# Autodesk Inventor assembly: Assembly2
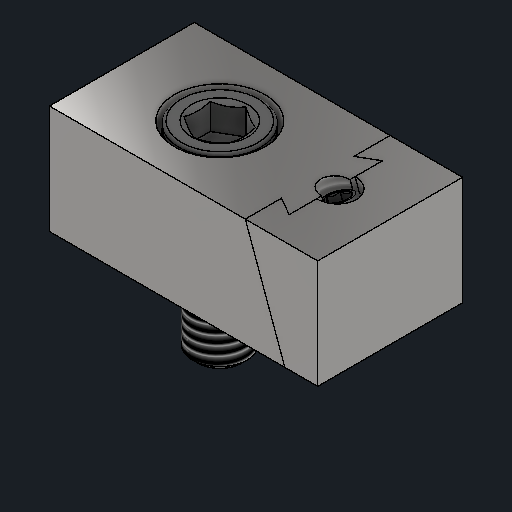
[picture p0: Inventor's stored thumbnail of the model, 512x512]
Saved by Autodesk Inventor 2026.2 (Build 302298000, 298)
## iProperties
Created: 2026-09-23
Part Number: Assembly2
Document SubType Name: Assembly
Designer: JoshuaEah
Author: JoshuaEah
## Documents named in this file (5)
- C:\Users\JoshuaEah\Documents\GitHub\Designed-Trinkets\Toe Clamps\Assembly2.iam
- C:\Users\JoshuaEah\Documents\GitHub\Designed-Trinkets\Toe Clamps\Part1.ipt
- C:\Users\JoshuaEah\Documents\GitHub\Designed-Trinkets\Toe Clamps\Part2.ipt
- C:\Users\JoshuaEah\Documents\GitHub\Designed-Trinkets\Toe Clamps\0.25-20x0.5 Set Screw.ipt
- C:\Users\JoshuaEah\Documents\GitHub\Designed-Trinkets\Toe Clamps\3-8-16x1 SHCS.ipt
## Components (4 placed, 4 different names)
1. Part1:1 — Slider:1, Insert:2
2. Part2:1 — Slider:1, Insert:1
3. 0.25-20x0.5 Set Screw:1 — Insert:1
4. 3-8-16x1 SHCS:1 — Insert:2
## Relationships (3: Insert 2, TranslationJoint 1)
- Slider:1 [TranslationJoint]: Part1:1 ↔ Part2:1
- Insert:1: Part2:1 ↔ 0.25-20x0.5 Set Screw:1
- Insert:2: Part1:1 ↔ 3-8-16x1 SHCS:1
